# Autodesk Inventor assembly: PIEZA4_COMPLETA
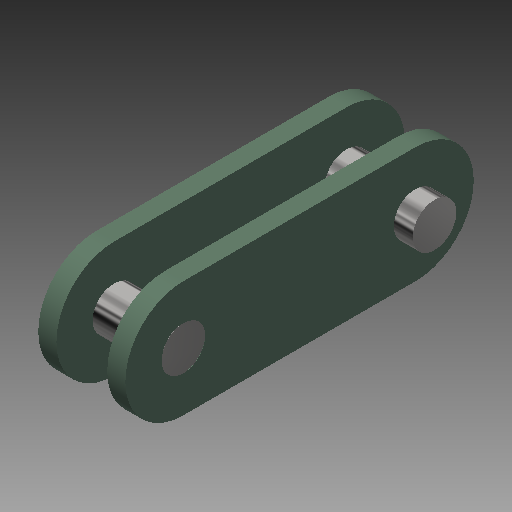
[picture p0: Inventor's stored thumbnail of the model, 512x512]
Saved by Autodesk Inventor 2019 (Build 230136000, 136)
## iProperties
Created: 2018-10-25
Part Number: PIEZA4_COMPLETA
Document SubType Name: Assembly
Designer: Isaac
Author: Isaac
## Documents named in this file (4)
- F:\BILBAO\CADCAM\LABORATORIO\BRIDA DE APRIETE\PIEZA4_COMPLETA.iam
- F:\BILBAO\CADCAM\LABORATORIO\BRIDA DE APRIETE\Part4.ipt
- F:\BILBAO\CADCAM\LABORATORIO\BRIDA DE APRIETE\Part4_PASADOR12.ipt
- F:\BILBAO\CADCAM\LABORATORIO\BRIDA DE APRIETE\Part4_PASADOR17.2.ipt
## Components (4 placed, 3 different names)
1. Part4:1 — Insert:1, Mate:2, Flush:1
2. Part4:2 — Insert:2, Mate:1
3. Part4_PASADOR12:2 — Insert:1, Insert:2
4. Part4_PASADOR17.2:1 — Mate:1, Mate:2, Flush:1
## Relationships (5: Insert 2, Mate 2, Flush 1)
- Insert:1: Part4:1 ↔ Part4_PASADOR12:2
- Insert:2: Part4:2 ↔ Part4_PASADOR12:2
- Mate:1: Part4:2 ↔ Part4_PASADOR17.2:1
- Mate:2: Part4:1 ↔ Part4_PASADOR17.2:1
- Flush:1 (-2.6 mm): Part4:1 ↔ Part4_PASADOR17.2:1
